# Autodesk Inventor assembly: High Strength 84-Tooth Gear, Square Insert
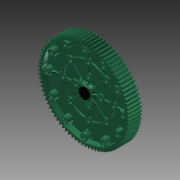
[picture p0: Inventor's stored thumbnail of the model, 180x180]
Saved by Autodesk Inventor 2015 (Build 190159000, 159)
## iProperties
Company: Bots 'n' Stuff
Created: 2014-06-27
Document SubType Name: Assembly
Designer: Jordan Kiesel
Vendor: VEX Robotics, Inc.
Mass: 43.5374 g
Surface Area: 282.615 cm^2
Volume: 28.725 cm^3
Density: 1.51566 g/cm^3
Author: Jordan Kiesel
Title: High Strength 84-Tooth Gear, Square Insert
## Documents named in this file (3)
- C:\Users\Jordan\Documents\CAD\2015 BNS CAD Library (beta)\Motion\Spur Gears\High Strength 84-Tooth Gear, Square Insert.iam
- C:\Users\Jordan\Documents\CAD\2015 BNS CAD Library (beta)\Motion\Spur Gears\Reference Parts\High Strength Gears\High Strength 84-Tooth Gear.ipt
- C:\Users\Jordan\Documents\CAD\2015 BNS CAD Library (beta)\Motion\Reference Parts\High Strength Square Gear Insert.ipt
## Components (3 placed, 2 different names)
1. High Strength 84-Tooth Gear:1 — Mate:1, Mate:2, Mate:3, Mate:4, Mate:5, Mate:6
2. High Strength Square Gear Insert:1 — Mate:1, Mate:2, Mate:3
3. High Strength Square Gear Insert:2 — Mate:4, Mate:5, Mate:6
## Relationships (6: Mate 6)
- Mate:1 (0.0254 mm): High Strength 84-Tooth Gear:1 ↔ High Strength Square Gear Insert:1
- Mate:2 (0.0254 mm): High Strength 84-Tooth Gear:1 ↔ High Strength Square Gear Insert:1
- Mate:3: High Strength 84-Tooth Gear:1 ↔ High Strength Square Gear Insert:1
- Mate:4 (0.0254 mm): High Strength 84-Tooth Gear:1 ↔ High Strength Square Gear Insert:2
- Mate:5 (0.0254 mm): High Strength 84-Tooth Gear:1 ↔ High Strength Square Gear Insert:2
- Mate:6: High Strength 84-Tooth Gear:1 ↔ High Strength Square Gear Insert:2
